# Autodesk Inventor assembly: linear drive
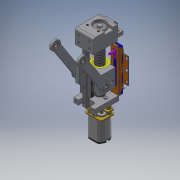
[picture p0: Inventor's stored thumbnail of the model, 180x180]
Saved by Autodesk Inventor 2017 (Build 210142000, 142)
## iProperties
Created: 2018-09-03
Part Number: linear drive
Document SubType Name: Assembly
Designer: Tomasz
Author: Tomasz
## Documents named in this file (16)
- C:\InventorVault-Lider\LiderWorkspace\LiderHand\linear drive\linear drive.iam
- C:\InventorVault-Lider\LiderWorkspace\LiderHand\linear drive\mount_front_side.ipt
- C:\InventorVault-Lider\LiderWorkspace\LiderHand\parts\DIN 988 - 4 x 8 x 0,1.ipt
- C:\InventorVault-Lider\LiderWorkspace\LiderHand\parts\bearing_thrust_3x8x3,5.ipt
- C:\InventorVault-Lider\LiderWorkspace\LiderHand\linear drive\igus_6.35x2.54_screw.ipt
- C:\InventorVault-Lider\LiderWorkspace\LiderHand\linear drive\mount_motor_side.ipt
- C:\InventorVault-Lider\LiderWorkspace\LiderHand\parts\micro-metal-gearmotor-standard-with-pinhole.ipt
- C:\InventorVault-Lider\LiderWorkspace\LiderHand\parts\igus_6.35x2.54_nut.ipt
- C:\InventorVault-Lider\LiderWorkspace\LiderHand\linear drive\trolley.ipt
- C:\InventorVault-Lider\LiderWorkspace\LiderHand\parts\wobit_rail_3ML-SS-block.ipt
- C:\InventorVault-Lider\LiderWorkspace\LiderHand\parts\wobit_rail_3M_lindrive.ipt
- C:\InventorVault-Lider\LiderWorkspace\LiderHand\linear drive\trolley_tendon_long_shaft.ipt
- C:\InventorVault-Lider\LiderWorkspace\LiderHand\parts\DIN 125 - A 2,2.ipt
- C:\InventorVault-Lider\LiderWorkspace\LiderHand\linear drive\tendon.ipt
- C:\InventorVault-Lider\LiderWorkspace\LiderHand\parts\bearing_2x5x1,5.ipt
- C:\InventorVault-Lider\LiderWorkspace\LiderHand\parts\alps_RDC1022A05.ipt
## Components (22 placed, 15 different names)
1. mount_front_side:1 — Flush:1, Mate:1, Mate:2, Mate:3, Mate:4, Mate:5, Mate:6, Mate:7, Mate:9, Mate:12, Mate:23, Flush:7, Mate:40, Flush:8
2. DIN 988 4 x 8 x 0,1:1 — Mate:3, Mate:4, Mate:8
3. DIN 988 4 x 8 x 0,1:2 — Mate:5, Mate:6, Mate:10
4. bearing_thrust_3x8x3,5:1 — Mate:7, Mate:8
5. bearing_thrust_3x8x3,5:2 — Mate:9, Mate:10, Mate:11
6. igus_6.35x2.54_screw:1 — Mate:11, Mate:12, Mate:17, Mate:25, Mate:41
7. mount_motor_side:1 — Mate:13, Mate:14, Mate:15, Mate:16
8. micro-metal-gearmotor-standard-with-pinhole:1 — Mate:14, Mate:15, Mate:16, Mate:17, Mate:41
9. igus_6.35x2.54_nut:1 — Mate:21, Mate:22, Mate:25
10. trolley:1 — Mate:18, Mate:19, Mate:20, Mate:21, Mate:22, Mate:27, Flush:2, Mate:30, Mate:31
11. wobit_rail_3ML-SS-block:1 — Mate:18, Mate:19, Mate:20, Mate:26
12. wobit_rail_3M_lindrive:1 — Mate:23, Mate:24, Mate:26
13. trolley_tendon_long_shaft:1 — Mate:27, Flush:2, Mate:28, Mate:29, Mate:36, Mate:37
14. DIN 125-1 A A 2,2:1 — Mate:29, Mate:30, Mate:38
15. DIN 125-1 A A 2,2:2 — Mate:28, Mate:31, Mate:39
16. tendon:1 — Mate:32, Mate:34, Flush:3, Flush:4, Angle:1
17. tendon:2 — Mate:33, Mate:35, Flush:5, Flush:6, Angle:1
18. bearing_2x5x1,5:1 — Mate:32, Flush:3, Mate:37, Mate:38
19. bearing_2x5x1,5:2 — Mate:33, Flush:6, Mate:36, Mate:39
20. bearing_2x5x1,5:3 — Mate:34, Flush:4
21. bearing_2x5x1,5:4 — Mate:35, Flush:5
22. alps_RDC1022A05:1 — Flush:7, Mate:40, Flush:8
## Relationships (50: Mate 41, Flush 8, Angle 1)
- Flush:1: mount_front_side:1
- Mate:1: mount_front_side:1
- Mate:2: mount_front_side:1
- Mate:3: mount_front_side:1 ↔ DIN 988 4 x 8 x 0,1:1
- Mate:4: mount_front_side:1 ↔ DIN 988 4 x 8 x 0,1:1
- Mate:5: mount_front_side:1 ↔ DIN 988 4 x 8 x 0,1:2
- Mate:6: mount_front_side:1 ↔ DIN 988 4 x 8 x 0,1:2
- Mate:7: mount_front_side:1 ↔ bearing_thrust_3x8x3,5:1
- Mate:8: DIN 988 4 x 8 x 0,1:1 ↔ bearing_thrust_3x8x3,5:1
- Mate:9: mount_front_side:1 ↔ bearing_thrust_3x8x3,5:2
- Mate:10: DIN 988 4 x 8 x 0,1:2 ↔ bearing_thrust_3x8x3,5:2
- Mate:11: bearing_thrust_3x8x3,5:2 ↔ igus_6.35x2.54_screw:1
- Mate:12: mount_front_side:1 ↔ igus_6.35x2.54_screw:1
- Mate:13: mount_motor_side:1
- Mate:14: mount_motor_side:1 ↔ micro-metal-gearmotor-standard-with-pinhole:1
- Mate:15: mount_motor_side:1 ↔ micro-metal-gearmotor-standard-with-pinhole:1
- Mate:16: mount_motor_side:1 ↔ micro-metal-gearmotor-standard-with-pinhole:1
- Mate:17: igus_6.35x2.54_screw:1 ↔ micro-metal-gearmotor-standard-with-pinhole:1
- Mate:18: trolley:1 ↔ wobit_rail_3ML-SS-block:1
- Mate:19: trolley:1 ↔ wobit_rail_3ML-SS-block:1
- Mate:20: trolley:1 ↔ wobit_rail_3ML-SS-block:1
- Mate:21: igus_6.35x2.54_nut:1 ↔ trolley:1
- Mate:22: igus_6.35x2.54_nut:1 ↔ trolley:1
- Mate:23: mount_front_side:1 ↔ wobit_rail_3M_lindrive:1
- Mate:24: wobit_rail_3M_lindrive:1
- Mate:25: igus_6.35x2.54_screw:1 ↔ igus_6.35x2.54_nut:1
- Mate:26: wobit_rail_3ML-SS-block:1 ↔ wobit_rail_3M_lindrive:1
- Mate:27: trolley:1 ↔ trolley_tendon_long_shaft:1
- Flush:2 (-2.8 mm): trolley:1 ↔ trolley_tendon_long_shaft:1
- Mate:28: trolley_tendon_long_shaft:1 ↔ DIN 125-1 A A 2,2:2
- Mate:29: trolley_tendon_long_shaft:1 ↔ DIN 125-1 A A 2,2:1
- Mate:30: trolley:1 ↔ DIN 125-1 A A 2,2:1
- Mate:31: trolley:1 ↔ DIN 125-1 A A 2,2:2
- Mate:32: tendon:1 ↔ bearing_2x5x1,5:1
- Mate:33: tendon:2 ↔ bearing_2x5x1,5:2
- Mate:34: tendon:1 ↔ bearing_2x5x1,5:3
- Mate:35: tendon:2 ↔ bearing_2x5x1,5:4
- Flush:3: tendon:1 ↔ bearing_2x5x1,5:1
- Flush:4: tendon:1 ↔ bearing_2x5x1,5:3
- Flush:5: tendon:2 ↔ bearing_2x5x1,5:4
- Flush:6: tendon:2 ↔ bearing_2x5x1,5:2
- Mate:36: trolley_tendon_long_shaft:1 ↔ bearing_2x5x1,5:2
- Mate:37: trolley_tendon_long_shaft:1 ↔ bearing_2x5x1,5:1
- Mate:38: DIN 125-1 A A 2,2:1 ↔ bearing_2x5x1,5:1
- Mate:39: DIN 125-1 A A 2,2:2 ↔ bearing_2x5x1,5:2
- Angle:1 (-90 deg): tendon:1 ↔ tendon:2
- Flush:7 (-3.6 mm): mount_front_side:1 ↔ alps_RDC1022A05:1
- Mate:40 (6 mm): mount_front_side:1 ↔ alps_RDC1022A05:1
- Flush:8 (8 mm): mount_front_side:1 ↔ alps_RDC1022A05:1
- Mate:41: igus_6.35x2.54_screw:1 ↔ micro-metal-gearmotor-standard-with-pinhole:1
